# Autodesk Inventor assembly: каретка
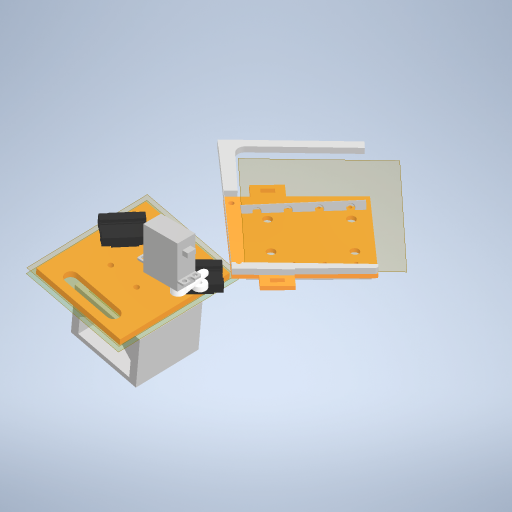
[picture p0: Inventor's stored thumbnail of the model, 512x512]
Saved by Autodesk Inventor 2024.2 (Build 282272000, 272)
## iProperties
Created: 1900-01-01
Part Number: каретка
Description: NONE
Document SubType Name: Assembly
Designer: Zakhar
Author: Zakhar
Revision Number: ANYUNSPECIFIED
## Documents named in this file (11)
- C:\Users\Service\Documents\Artist\3D\каретка.iam
- C:\Users\Service\Documents\Artist\3D\стл\Сборка плоттер\Сервопривод.ipt
- C:\Users\Service\Documents\Artist\3D\стл\Сборка плоттер\Пластина.ipt
- C:\Users\Service\Documents\Artist\3D\стл\Сборка плоттер\MGN7 rail_100 mm.ipt
- C:\Users\Service\Documents\Artist\3D\стл\Сборка плоттер\MGN7C_MGN7C.ipt
- C:\Users\Service\Documents\Artist\3D\стл\Сборка плоттер\Каретка-втулки.ipt
- C:\Users\Service\Documents\Artist\3D\стл\Сборка плоттер\Деталь.ipt
- C:\Users\Service\Documents\Artist\3D\стл\Сборка плоттер\Деталь_1.ipt
- C:\Users\Service\Documents\Artist\3D\соединялка.ipt
- C:\Users\Service\Documents\Artist\3D\стл\полное крепление каретки.ipt
- C:\Users\Service\Documents\Artist\3D\стл\верх крепления маркера.ipt
## Components (12 placed, 4 different names)
1. ANY
2. ANY:5 — Совмещение:7, Совмещение:8, Совмещение:9, Совмещение:10, Заподлицо:3, Заподлицо:4, Заподлицо:5
3. ANY:6 — Совмещение:1, Совмещение:2
4. ANY:7 — Совмещение:1, Совмещение:8, Совмещение:9
5. ANY:8 — Совмещение:3, Совмещение:4, Совмещение:5, Совмещение:6
6. ANY:9 — Совмещение:5, Совмещение:7, Совмещение:10
7. ANY:13 — Заподлицо:1, Заподлицо:2, Совмещение:2, Совмещение:3, Совмещение:4, Совмещение:6
8. ANY:14
9. ANY:15
10. соединялка:1 — Заподлицо:1, Заподлицо:2
11. полное крепление каретки:1 — Заподлицо:3, Заподлицо:4, Заподлицо:5, Заподлицо:6, Заподлицо:8
12. верх крепления маркера:1 — Заподлицо:6, Заподлицо:8
## Relationships (17: Mate 10, Flush 7)
- Заподлицо:1 [Flush]: ANY:13 ↔ соединялка:1
- Заподлицо:2 [Flush]: ANY:13 ↔ соединялка:1
- Совмещение:1 [Mate]: ANY:6 ↔ ANY:7
- Совмещение:2 [Mate]: ANY:6 ↔ ANY:13
- Совмещение:3 [Mate]: ANY:8 ↔ ANY:13
- Совмещение:4 [Mate]: ANY:8 ↔ ANY:13
- Совмещение:5 [Mate]: ANY:8 ↔ ANY:9
- Совмещение:6 [Mate]: ANY:8 ↔ ANY:13
- Совмещение:7 [Mate]: ANY:5 ↔ ANY:9
- Совмещение:8 [Mate]: ANY:5 ↔ ANY:7
- Совмещение:9 [Mate]: ANY:5 ↔ ANY:7
- Совмещение:10 [Mate]: ANY:5 ↔ ANY:9
- Заподлицо:3 [Flush]: ANY:5 ↔ полное крепление каретки:1
- Заподлицо:4 [Flush]: ANY:5 ↔ полное крепление каретки:1
- Заподлицо:5 [Flush]: ANY:5 ↔ полное крепление каретки:1
- Заподлицо:6 [Flush]: полное крепление каретки:1 ↔ верх крепления маркера:1
- Заподлицо:8 [Flush] (5 mm): полное крепление каретки:1 ↔ верх крепления маркера:1
